# Autodesk Inventor assembly: LucasCharles Assembly Final V2
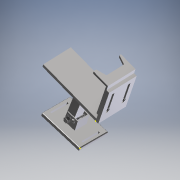
[picture p0: Inventor's stored thumbnail of the model, 180x180]
Saved by Autodesk Inventor 2018 (Build 220112000, 112)
## iProperties
Created: 2018-05-23
Part Number: LucasCharles Assembly Final V2
Document SubType Name: Assembly
Designer: 21lsilva
Author: 21lsilva
## Documents named in this file (12)
- \\Pluto\students\2021\21lsilva\I.E.D\Unit9\LucasCharles Assembly Final V2.iam
- \\Joker\students\2019\19cbaiden\Introduction to Engineering Design\LUCASCHARLES\FINAL\LucasCharles Part 1 wall mount FINAL v2.ipt
- \\Joker\students\2019\19cbaiden\Introduction to Engineering Design\LUCASCHARLES\FINAL\LucasCharles Part 2 arm Final.ipt
- \\Joker\students\2019\19cbaiden\Introduction to Engineering Design\LUCASCHARLES\FINAL\LucasCharles Part 4 bolt to hold arm to wall mount Final.ipt
- \\Joker\students\2019\19cbaiden\Introduction to Engineering Design\LUCASCHARLES\FINAL\LucasCharles part 5 nut final.ipt
- \\Joker\students\2019\19cbaiden\Introduction to Engineering Design\LUCASCHARLES\FINAL\LucasCharles Part 10 final.ipt
- \\Joker\students\2019\19cbaiden\Introduction to Engineering Design\LUCASCHARLES\FINAL\LucasCharles part11 final.ipt
- \\Joker\students\2019\19cbaiden\Introduction to Engineering Design\LUCASCHARLES\FINAL\LucasCharles Part6 bolt for arm to speaker holder Final.ipt
- \\Pluto\students\2021\21lsilva\I.E.D\Unit9\LucasCharles part 5 nut.ipt
- \\Pluto\students\2021\21lsilva\I.E.D\Unit9\LucasCharles Part 8 small nut.ipt
- \\Joker\students\2019\19cbaiden\Introduction to Engineering Design\LUCASCHARLES\FINAL\LucasCharles Part7 bolt for height Final.ipt
- \\Joker\students\2019\19cbaiden\Introduction to Engineering Design\LUCASCHARLES\FINAL\LucasCharles Part 8 small nut Final.ipt
## Components (12 placed, 11 different names)
1. LucasCharles Part 1 wall mount FINAL v2:1 — Mate:1, Mate:2, Mate:14, Mate:15, Mate:16, Mate:18, Mate:20
2. LucasCharles Part 10 final:1 — Mate:9, Flush:1, Mate:11, Mate:13
3. LucasCharles part11 final:1 — Mate:3, Mate:4, Mate:5, Mate:6, Mate:7, Mate:9, Flush:1, Mate:10, Mate:12
4. LucasCharles Part6 bolt for arm to speaker holder Final:1 — Mate:5, Mate:6, Mate:8
5. LucasCharles Part 2 arm Final:1 — Mate:1, Mate:2, Mate:3, Mate:4, Mate:17
6. LucasCharles part 5 nut:1 — Mate:7, Mate:8
7. LucasCharles Part 8 small nut:1 — Mate:12, Mate:13
8. LucasCharles Part 8 small nut:2 — Mate:10, Mate:11
9. LucasCharles Part7 bolt for height Final:1 — Mate:14, Mate:15, Mate:21
10. LucasCharles Part 4 bolt to hold arm to wall mount Final:1 — Mate:16, Mate:17, Mate:19
11. LucasCharles part 5 nut final:1 — Mate:18, Mate:19
12. LucasCharles Part 8 small nut Final:1 — Mate:20, Mate:21
## Relationships (22: Mate 21, Flush 1)
- Mate:1: LucasCharles Part 1 wall mount FINAL v2:1 ↔ LucasCharles Part 2 arm Final:1
- Mate:2: LucasCharles Part 1 wall mount FINAL v2:1 ↔ LucasCharles Part 2 arm Final:1
- Mate:3: LucasCharles part11 final:1 ↔ LucasCharles Part 2 arm Final:1
- Mate:4: LucasCharles part11 final:1 ↔ LucasCharles Part 2 arm Final:1
- Mate:5: LucasCharles part11 final:1 ↔ LucasCharles Part6 bolt for arm to speaker holder Final:1
- Mate:6: LucasCharles part11 final:1 ↔ LucasCharles Part6 bolt for arm to speaker holder Final:1
- Mate:7: LucasCharles part11 final:1 ↔ LucasCharles part 5 nut:1
- Mate:8: LucasCharles Part6 bolt for arm to speaker holder Final:1 ↔ LucasCharles part 5 nut:1
- Mate:9: LucasCharles Part 10 final:1 ↔ LucasCharles part11 final:1
- Flush:1: LucasCharles Part 10 final:1 ↔ LucasCharles part11 final:1
- Mate:10: LucasCharles part11 final:1 ↔ LucasCharles Part 8 small nut:2
- Mate:11: LucasCharles Part 10 final:1 ↔ LucasCharles Part 8 small nut:2
- Mate:12: LucasCharles part11 final:1 ↔ LucasCharles Part 8 small nut:1
- Mate:13: LucasCharles Part 10 final:1 ↔ LucasCharles Part 8 small nut:1
- Mate:14: LucasCharles Part 1 wall mount FINAL v2:1 ↔ LucasCharles Part7 bolt for height Final:1
- Mate:15: LucasCharles Part 1 wall mount FINAL v2:1 ↔ LucasCharles Part7 bolt for height Final:1
- Mate:16: LucasCharles Part 1 wall mount FINAL v2:1 ↔ LucasCharles Part 4 bolt to hold arm to wall mount Final:1
- Mate:17: LucasCharles Part 2 arm Final:1 ↔ LucasCharles Part 4 bolt to hold arm to wall mount Final:1
- Mate:18: LucasCharles Part 1 wall mount FINAL v2:1 ↔ LucasCharles part 5 nut final:1
- Mate:19: LucasCharles Part 4 bolt to hold arm to wall mount Final:1 ↔ LucasCharles part 5 nut final:1
- Mate:20: LucasCharles Part 1 wall mount FINAL v2:1 ↔ LucasCharles Part 8 small nut Final:1
- Mate:21: LucasCharles Part7 bolt for height Final:1 ↔ LucasCharles Part 8 small nut Final:1
